# Autodesk Inventor assembly: Inner Channel
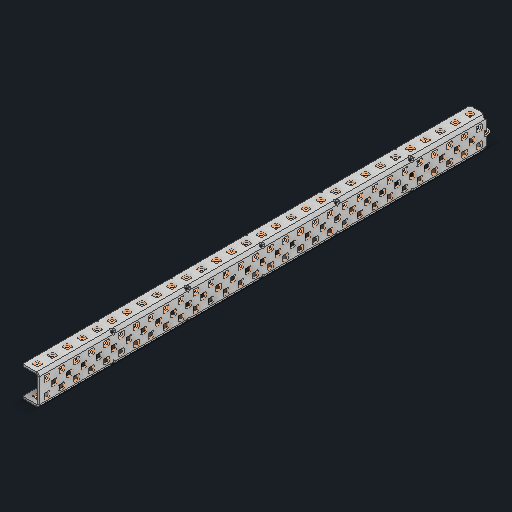
[picture p0: Inventor's stored thumbnail of the model, 512x512]
Saved by Autodesk Inventor 2025.1 (Build 291241000, 241)
## iProperties
Created: 2024-11-04
Part Number: Inner Channel
Document SubType Name: Assembly
Designer: avere
Author: avere
## Documents named in this file (2)
- C:\Users\avere\VEX\High Stakes\CAD\V3\Chassis\Drivebay Left\Inner Channel.iam
- C:\Users\avere\VEX\High Stakes\CAD\ROBOPROS-CAD-Inventor\Structure\C Channel\Aluminum 1x2x1\Alu C 1x2x1x30.ipt
## Components (1 placed, 1 different names)
1. Alu C 1x2x1x30:1 — Flush:1, Flush:2, Flush:3
## Relationships (3: Flush 3)
- Flush:1 (-190.5 mm): Alu C 1x2x1x30:1
- Flush:2 (-7.9375 mm): Alu C 1x2x1x30:1
- Flush:3 (-12.7 mm): Alu C 1x2x1x30:1
